# Autodesk Inventor assembly: frame
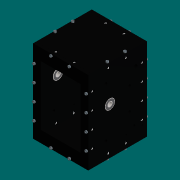
[picture p0: Inventor's stored thumbnail of the model, 180x180]
Saved by Autodesk Inventor 2016 (Build 200138000, 138)
## iProperties
Created: 2015-10-05
Part Number: frame
Document SubType Name: Assembly
Designer: Sawaiz
Author: Sawaiz
## Documents named in this file (7)
- C:\Users\sawai\OneDrive\projects\splitFlapDisplay\frame\frame.iam
- C:\Users\sawai\OneDrive\projects\splitFlapDisplay\frame\front.ipt
- C:\Users\sawai\OneDrive\projects\splitFlapDisplay\frame\back.ipt
- C:\Users\sawai\OneDrive\projects\splitFlapDisplay\frame\side.ipt
- C:\Users\sawai\OneDrive\projects\splitFlapDisplay\frame\topBottomPanel.ipt
- C:\Users\sawai\OneDrive\projects\splitFlapDisplay\frame\608RS.ipt
- C:\Users\sawai\OneDrive\projects\splitFlapDisplay\frame\panelScrewNut.iam
## Components (40 placed, 6 different names)
1. front:1 — Mate:1, Flush:1, Flush:2, Mate:2, Flush:4, Mate:4, Flush:5, Mate:6, Mate:11, Mate:12, Mate:13, Mate:14, Mate:15, Mate:16, Mate:17, Mate:18, Mate:19, Mate:20, Mate:25, Mate:26, Angle:12, Mate:43
2. back:1 — Mate:1, Flush:1, Flush:3, Mate:3, Flush:6, Mate:7, Mate:27, Mate:28, Mate:29, Mate:30, Mate:31, Mate:32, Mate:33, Mate:34, Mate:35, Mate:36, Mate:37, Mate:38, Angle:34, Mate:46
3. side:1 — Flush:7, Mate:7, Mate:8, Mate:10, Flush:9
4. topBottomPanel:1 — Flush:2, Mate:2, Flush:3, Mate:3, Mate:5, Flush:7, Mate:8, Mate:21, Mate:22, Mate:23, Mate:24, Mate:45, Angle:35
5. side:2 — Flush:6, Mate:5, Mate:6, Mate:9, Flush:8
6. topBottomPanel:2 — Flush:4, Mate:4, Flush:5, Mate:39, Mate:40, Mate:41, Mate:42, Angle:20, Mate:44
7. 608RS:1 — Mate:10, Flush:9
8. 608RS:2 — Mate:9, Flush:8
9. panelScrewNut:1 [sub-assembly] — Mate:42, Flush:37, Angle:17, Angle:18
10. panelScrewNut:2 [sub-assembly] — Mate:11, Flush:20, Angle:1
11. panelScrewNut:3 [sub-assembly] — Mate:12, Flush:18, Flush:19, Angle:2, Angle:3
12. panelScrewNut:4 [sub-assembly] — Mate:21, Flush:32, Angle:15
13. panelScrewNut:5 [sub-assembly] — Mate:34, Flush:24, Flush:25, Angle:27, Angle:28
14. panelScrewNut:6 [sub-assembly] — Mate:16, Flush:16, Flush:17, Angle:4, Angle:5
15. panelScrewNut:7 [sub-assembly] — Mate:40, Flush:35, Angle:19, Angle:20
16. panelScrewNut:8 [sub-assembly] — Mate:25, Flush:10, Flush:11, Angle:10, Angle:11, Mate:43
17. panelScrewNut:9 [sub-assembly] — Mate:14, Flush:19, Flush:20, Angle:1, Angle:2
18. panelScrewNut:10 [sub-assembly] — Mate:41, Flush:36, Flush:37, Angle:17, Mate:44
19. panelScrewNut:11 [sub-assembly] — Mate:23, Flush:34, Angle:13, Mate:45, Angle:35
20. panelScrewNut:12 [sub-assembly] — Mate:39, Flush:35, Flush:36, Angle:18, Angle:19
21. panelScrewNut:13 [sub-assembly] — Mate:22, Flush:32, Flush:33, Angle:14, Angle:15
22. panelScrewNut:14 [sub-assembly] — Mate:24, Flush:33, Flush:34, Angle:13, Angle:14
23. panelScrewNut:15 [sub-assembly] — Mate:36, Flush:22, Flush:23, Angle:29, Angle:30
24. panelScrewNut:16 [sub-assembly] — Mate:32, Flush:26, Flush:27, Angle:25, Angle:26
25. panelScrewNut:17 [sub-assembly] — Mate:28, Flush:30, Flush:31, Angle:21, Angle:34, Mate:46
26. panelScrewNut:18 [sub-assembly] — Mate:29, Flush:29, Flush:30, Angle:23
27. panelScrewNut:19 [sub-assembly] — Mate:26, Flush:10, Angle:11, Angle:12
28. panelScrewNut:20 [sub-assembly] — Mate:31, Flush:27, Flush:28, Angle:24, Angle:25
29. panelScrewNut:21 [sub-assembly] — Mate:35, Flush:23, Flush:24, Angle:28, Angle:29
30. panelScrewNut:22 [sub-assembly] — Mate:33, Flush:25, Flush:26, Angle:26, Angle:27
31. panelScrewNut:23 [sub-assembly] — Mate:30, Flush:28, Flush:29, Angle:23, Angle:24
32. panelScrewNut:24 [sub-assembly] — Mate:20, Flush:11, Flush:12, Angle:9, Angle:10
33. panelScrewNut:25 [sub-assembly] — Mate:27, Flush:31, Angle:21, Angle:32
34. panelScrewNut:26 [sub-assembly] — Mate:37, Flush:21, Flush:22, Angle:30, Angle:31
35. panelScrewNut:27 [sub-assembly] — Mate:38, Flush:21, Angle:31, Angle:32
36. panelScrewNut:28 [sub-assembly] — Mate:19, Flush:12, Flush:13, Angle:8, Angle:9
37. panelScrewNut:29 [sub-assembly] — Mate:17, Flush:14, Flush:15, Angle:6, Angle:7
38. panelScrewNut:30 [sub-assembly] — Mate:18, Flush:13, Flush:14, Angle:7, Angle:8
39. panelScrewNut:31 [sub-assembly] — Mate:13, Flush:17, Flush:18, Angle:3, Angle:4
40. panelScrewNut:32 [sub-assembly] — Mate:15, Flush:15, Flush:16, Angle:5, Angle:6
## Relationships (115: Mate 46, Flush 37, Angle 32)
- Mate:1: front:1 ↔ back:1
- Flush:1: front:1 ↔ back:1
- Flush:2: front:1 ↔ topBottomPanel:1
- Mate:2: front:1 ↔ topBottomPanel:1
- Flush:3: back:1 ↔ topBottomPanel:1
- Mate:3: back:1 ↔ topBottomPanel:1
- Flush:4: front:1 ↔ topBottomPanel:2
- Mate:4: front:1 ↔ topBottomPanel:2
- Flush:5: front:1 ↔ topBottomPanel:2
- Flush:6: back:1 ↔ side:2
- Mate:5: topBottomPanel:1 ↔ side:2
- Mate:6: front:1 ↔ side:2
- Flush:7: side:1 ↔ topBottomPanel:1
- Mate:7: back:1 ↔ side:1
- Mate:8: side:1 ↔ topBottomPanel:1
- Mate:9: side:2 ↔ 608RS:2
- Flush:8: side:2 ↔ 608RS:2
- Mate:10: side:1 ↔ 608RS:1
- Flush:9: side:1 ↔ 608RS:1
- Mate:11: front:1 ↔ panelScrewNut:2
- Mate:12: front:1 ↔ panelScrewNut:3
- Mate:13: front:1 ↔ panelScrewNut:31
- Mate:14: front:1 ↔ panelScrewNut:9
- Mate:15: front:1 ↔ panelScrewNut:32
- Mate:16: front:1 ↔ panelScrewNut:6
- Mate:17: front:1 ↔ panelScrewNut:29
- Mate:18: front:1 ↔ panelScrewNut:30
- Mate:19: front:1 ↔ panelScrewNut:28
- Mate:20: front:1 ↔ panelScrewNut:24
- Mate:21: topBottomPanel:1 ↔ panelScrewNut:4
- Mate:22: topBottomPanel:1 ↔ panelScrewNut:13
- Mate:23: topBottomPanel:1 ↔ panelScrewNut:11
- Mate:24: topBottomPanel:1 ↔ panelScrewNut:14
- Mate:25: front:1 ↔ panelScrewNut:8
- Mate:26: front:1 ↔ panelScrewNut:19
- Mate:27: back:1 ↔ panelScrewNut:25
- Mate:28: back:1 ↔ panelScrewNut:17
- Mate:29: back:1 ↔ panelScrewNut:18
- Mate:30: back:1 ↔ panelScrewNut:23
- Mate:31: back:1 ↔ panelScrewNut:20
- Mate:32: back:1 ↔ panelScrewNut:16
- Mate:33: back:1 ↔ panelScrewNut:22
- Mate:34: back:1 ↔ panelScrewNut:5
- Mate:35: back:1 ↔ panelScrewNut:21
- Mate:36: back:1 ↔ panelScrewNut:15
- Mate:37: back:1 ↔ panelScrewNut:26
- Mate:38: back:1 ↔ panelScrewNut:27
- Mate:39: topBottomPanel:2 ↔ panelScrewNut:12
- Mate:40: topBottomPanel:2 ↔ panelScrewNut:7
- Mate:41: topBottomPanel:2 ↔ panelScrewNut:10
- Mate:42: topBottomPanel:2 ↔ panelScrewNut:1
- Flush:10: panelScrewNut:8 ↔ panelScrewNut:19
- Flush:11: panelScrewNut:8 ↔ panelScrewNut:24
- Flush:12: panelScrewNut:24 ↔ panelScrewNut:28
- Flush:13: panelScrewNut:28 ↔ panelScrewNut:30
- Flush:14: panelScrewNut:29 ↔ panelScrewNut:30
- Flush:15: panelScrewNut:29 ↔ panelScrewNut:32
- Flush:16: panelScrewNut:6 ↔ panelScrewNut:32
- Flush:17: panelScrewNut:6 ↔ panelScrewNut:31
- Flush:18: panelScrewNut:3 ↔ panelScrewNut:31
- Flush:19: panelScrewNut:3 ↔ panelScrewNut:9
- Flush:20: panelScrewNut:2 ↔ panelScrewNut:9
- Flush:21: panelScrewNut:26 ↔ panelScrewNut:27
- Flush:22: panelScrewNut:15 ↔ panelScrewNut:26
- Flush:23: panelScrewNut:15 ↔ panelScrewNut:21
- Flush:24: panelScrewNut:5 ↔ panelScrewNut:21
- Flush:25: panelScrewNut:5 ↔ panelScrewNut:22
- Flush:26: panelScrewNut:16 ↔ panelScrewNut:22
- Flush:27: panelScrewNut:16 ↔ panelScrewNut:20
- Flush:28: panelScrewNut:20 ↔ panelScrewNut:23
- Flush:29: panelScrewNut:18 ↔ panelScrewNut:23
- Flush:30: panelScrewNut:17 ↔ panelScrewNut:18
- Flush:31: panelScrewNut:17 ↔ panelScrewNut:25
- Flush:32: panelScrewNut:4 ↔ panelScrewNut:13
- Flush:33: panelScrewNut:13 ↔ panelScrewNut:14
- Flush:34: panelScrewNut:11 ↔ panelScrewNut:14
- Flush:35: panelScrewNut:7 ↔ panelScrewNut:12
- Flush:36: panelScrewNut:10 ↔ panelScrewNut:12
- Flush:37: panelScrewNut:1 ↔ panelScrewNut:10
- Angle:1 (0 deg): panelScrewNut:2 ↔ panelScrewNut:9
- Angle:2 (0 deg): panelScrewNut:3 ↔ panelScrewNut:9
- Angle:3 (0 deg): panelScrewNut:3 ↔ panelScrewNut:31
- Angle:4 (90 deg): panelScrewNut:6 ↔ panelScrewNut:31
- Angle:5 (0 deg): panelScrewNut:6 ↔ panelScrewNut:32
- Angle:6 (90 deg): panelScrewNut:29 ↔ panelScrewNut:32
- Angle:7 (0 deg): panelScrewNut:29 ↔ panelScrewNut:30
- Angle:8 (0 deg): panelScrewNut:28 ↔ panelScrewNut:30
- Angle:9 (0 deg): panelScrewNut:24 ↔ panelScrewNut:28
- Angle:10 (90 deg): panelScrewNut:8 ↔ panelScrewNut:24
- Angle:11 (0 deg): panelScrewNut:8 ↔ panelScrewNut:19
- Angle:12 (0 deg): front:1 ↔ panelScrewNut:19
- Mate:43: front:1 ↔ panelScrewNut:8
- Angle:13 (0 deg): panelScrewNut:11 ↔ panelScrewNut:14
- Angle:14 (0 deg): panelScrewNut:13 ↔ panelScrewNut:14
- Angle:15 (0 deg): panelScrewNut:4 ↔ panelScrewNut:13
- Angle:17 (0 deg): panelScrewNut:1 ↔ panelScrewNut:10
- Angle:18 (0 deg): panelScrewNut:1 ↔ panelScrewNut:12
- Angle:19 (0 deg): panelScrewNut:7 ↔ panelScrewNut:12
- Angle:20 (90 deg): topBottomPanel:2 ↔ panelScrewNut:7
- Mate:44: topBottomPanel:2 ↔ panelScrewNut:10
- Mate:45: topBottomPanel:1 ↔ panelScrewNut:11
- Angle:21 (0 deg): panelScrewNut:17 ↔ panelScrewNut:25
- Angle:23 (0 deg): panelScrewNut:18 ↔ panelScrewNut:23
- Angle:24 (0 deg): panelScrewNut:20 ↔ panelScrewNut:23
- Angle:25 (0 deg): panelScrewNut:16 ↔ panelScrewNut:20
- Angle:26 (90 deg): panelScrewNut:16 ↔ panelScrewNut:22
- Angle:27 (0 deg): panelScrewNut:5 ↔ panelScrewNut:22
- Angle:28 (90 deg): panelScrewNut:5 ↔ panelScrewNut:21
- Angle:29 (0 deg): panelScrewNut:15 ↔ panelScrewNut:21
- Angle:30 (0 deg): panelScrewNut:15 ↔ panelScrewNut:26
- Angle:31 (0 deg): panelScrewNut:26 ↔ panelScrewNut:27
- Angle:32 (90 deg): panelScrewNut:25 ↔ panelScrewNut:27
- Angle:34 (0 deg): back:1 ↔ panelScrewNut:17
- Mate:46: back:1 ↔ panelScrewNut:17
- Angle:35 (90 deg): topBottomPanel:1 ↔ panelScrewNut:11
